# Autodesk Inventor assembly: Central Assembly
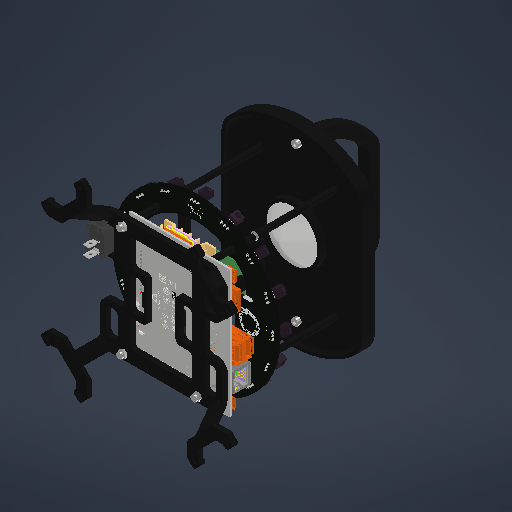
[picture p0: Inventor's stored thumbnail of the model, 512x512]
Saved by Autodesk Inventor 2026.1 (Build 301233020, 233B)
## iProperties
Created: 2026-04-06
Part Number: Central Assembly
Document SubType Name: Assembly
Designer: Bahaa
Mass: 258.249 g
Surface Area: 2094.89 cm^2
Volume: 209.179 cm^3
Density: 1.23458 g/cm^3
Author: Bahaa
## iProperties of the stored document MemberDocs/xZmzij4b1AkjbufniLng3pczf1d
Created: 2026-04-06
Part Number: Central Assembly
Document SubType Name: Assembly
Designer: Bahaa
Mass: 258.233 g
Surface Area: 2094.99 cm^2
Volume: 209.164 cm^3
Density: 1.2346 g/cm^3
Author: Bahaa
## Documents named in this file (20)
- C:\Users\Bahaa\Nextcloud2\CAD\25-26\V2\Central Assembly.iam
- C:\Users\Bahaa\Nextcloud2\CAD\25-26\V2\Center Hub.ipt
- C:\Users\Bahaa\Nextcloud2\CAD\25-26\V2\Parts\675_13541_batuu_dev_kit_top_ass_asm\675_13541_batuu_dev_kit_top_ass_asm.iam
- C:\Users\Bahaa\Nextcloud2\CAD\25-26\V2\Parts\R13-66A-02-BB2.ipt
- C:\Users\Bahaa\Nextcloud2\CAD\25-26\V2\Threaded Rod.ipt
- C:\Users\Bahaa\Documents\Inventor\Content Center Files\R2026\en-US\DIN 985\DIN 985 - M3.ipt
- C:\Users\Bahaa\Documents\Inventor\Content Center Files\R2026\en-US\DIN 934\DIN 934 - M2,5 x 0,45.ipt
- C:\Users\Bahaa\Nextcloud2\CAD\25-26\V2\Rod Housing Jetson.ipt
- C:\Users\Bahaa\Nextcloud2\CAD\25-26\V2\Rod Housing Cam.ipt
- C:\Users\Bahaa\Nextcloud2\CAD\25-26\V2\Camera Bracket.ipt
- C:\Users\Bahaa\Nextcloud2\CAD\25-26\V2\Parts\Kamera.ipt
- C:\Users\Bahaa\Nextcloud2\CAD\25-26\V2\Rod Housing Mirror.ipt
- C:\Users\Bahaa\Nextcloud2\CAD\25-26\V2\Top Cover.ipt
- C:\Users\Bahaa\Nextcloud2\CAD\25-26\V2\Mirror.ipt
- C:\Users\Bahaa\Nextcloud2\CAD\25-26\V2\Handle.ipt
- C:\Users\Bahaa\Documents\Inventor\Content Center Files\R2026\en-US\DIN 912\DIN 912 - M1,6 x 0,35 x 2,5 x 1,625.ipt
- C:\Users\Bahaa\Documents\Inventor\Content Center Files\R2026\en-US\DIN 912\DIN 912 - M3 x 0,5 x 5 x 3,75.ipt
- C:\Users\Bahaa\Nextcloud2\CAD\25-26\V2\Magnet 10x3x2mm.ipt
- C:\Users\Bahaa\Nextcloud2\CAD\25-26\V2\Tag.ipt
- C:\Users\Bahaa\Nextcloud2\CAD\25-26\V2\Boards\IR Board\IR Board\IR Board.iam
## Components (54 placed, 19 different names)
1. Center Hub:1 — Mate:2, Mate:3, Mate:4, Mate:5, Mate:6, Mate:7, Insert:1, Insert:2, Insert:3, Insert:4, Mate:8, Mate:9, Insert:5, Insert:6, Insert:7, Insert:8
2. Camera Bracket:1 — Mate:31, Mate:32, Mate:33, Mate:34, Mate:35, Mate:36, Mate:38, Mate:40, Mate:42, Mate:44
3. Top Cover:1 — Mate:45, Mate:48, Mate:49, Mate:50, Mate:51, Mate:52, Mate:53, Mate:54, Mate:55, Insert:25, Insert:26, Insert:27, Insert:28, Insert:29, Insert:30, Insert:31, Insert:32, Mate:56, Mate:57, Mate:58, Mate:59, Mate:60, Mate:61, Flush:5, Flush:6, Mate:68
4. Handle:1 — Mate:50, Mate:53, Mate:54, Mate:55
5. Mirror:1 — Mate:48, Mate:49
6. Tag:1 — Mate:62, Mate:63, Mate:64, Mate:65, Mate:66, Mate:67, Flush:5, Flush:6, Mate:68
7. IR Board:1 [sub-assembly] — Mate:69, Mate:70, Mate:71
8. Magnet 10x3x2mm:4 — Mate:62, Mate:66, Mate:67
9. Magnet 10x3x2mm:3 — Mate:63, Mate:64, Mate:65
10. Magnet 10x3x2mm:2 — Mate:59, Mate:60, Mate:61
11. Magnet 10x3x2mm:1 — Mate:56, Mate:57, Mate:58
12. DIN 985 - replaced by DIN EN ISO 10511 M3:8 — Insert:32
13. DIN 985 - replaced by DIN EN ISO 10511 M3:7 — Insert:31
14. DIN 985 - replaced by DIN EN ISO 10511 M3:6 — Insert:30
15. DIN 985 - replaced by DIN EN ISO 10511 M3:5 — Insert:29
16. DIN 912 - replaced by DIN EN ISO 4762 M3 x 5:4 — Insert:28
17. DIN 912 - replaced by DIN EN ISO 4762 M3 x 5:3 — Insert:27
18. DIN 912 - replaced by DIN EN ISO 4762 M3 x 5:2 — Insert:26
19. DIN 912 - replaced by DIN EN ISO 4762 M3 x 5:1 — Insert:25
20. DIN 912 - replaced by DIN EN ISO 4762 M1,6 x 2,5:4 — Insert:24
21. DIN 912 - replaced by DIN EN ISO 4762 M1,6 x 2,5:3 — Insert:23
22. DIN 912 - replaced by DIN EN ISO 4762 M1,6 x 2,5:2 — Insert:22
23. DIN 912 - replaced by DIN EN ISO 4762 M1,6 x 2,5:1 — Insert:21
24. DIN 934 - replaced by DIN EN 24032/28673/28674 M2,5:8 — Insert:12
25. DIN 934 - replaced by DIN EN 24032/28673/28674 M2,5:7 — Insert:11, Mate:32
26. DIN 934 - replaced by DIN EN 24032/28673/28674 M2,5:6 — Insert:10
27. DIN 934 - replaced by DIN EN 24032/28673/28674 M2,5:5 — Insert:9
28. DIN 934 - replaced by DIN EN 24032/28673/28674 M2,5:4 — Insert:8
29. DIN 934 - replaced by DIN EN 24032/28673/28674 M2,5:3 — Insert:7, Mate:11
30. DIN 934 - replaced by DIN EN 24032/28673/28674 M2,5:2 — Insert:6
31. DIN 934 - replaced by DIN EN 24032/28673/28674 M2,5:1 — Insert:5
32. DIN 985 - replaced by DIN EN ISO 10511 M3:1 — Insert:1, Flush:2
33. DIN 985 - replaced by DIN EN ISO 10511 M3:2 — Insert:2, Flush:3
34. DIN 985 - replaced by DIN EN ISO 10511 M3:3 — Insert:3, Mate:10, Flush:4
35. DIN 985 - replaced by DIN EN ISO 10511 M3:4 — Insert:4, Flush:1
36. Threaded Rod:1 — Mate:7, Flush:2, Mate:18, Mate:27, Mate:39, Mate:70
37. Threaded Rod:2 — Mate:8, Flush:1, Mate:12, Mate:29, Mate:31, Mate:41, Mate:51
38. Threaded Rod:3 — Mate:9, Flush:3, Mate:19, Mate:22, Mate:28, Mate:37, Mate:52, Mate:71
39. Threaded Rod:4 — Mate:10, Flush:4, Mate:17, Mate:30, Mate:33, Mate:43
40. Rod Housing Mirror:1 — Mate:37, Mate:38
41. Rod Housing Mirror:2 — Mate:39, Mate:40
42. Rod Housing Mirror:3 — Mate:41, Mate:42
43. Rod Housing Mirror:4 — Mate:43, Mate:44, Mate:45
44. Rod Housing Cam:1 — Mate:27, Insert:9
45. Rod Housing Cam:2 — Mate:30, Insert:12
46. Rod Housing Cam:3 — Mate:29, Insert:11
47. Rod Housing Cam:4 — Mate:28, Insert:10
48. Rod Housing Jetson:2 — Mate:14, Mate:17
49. Rod Housing Jetson:3 — Mate:16, Mate:19, Mate:22
50. Rod Housing Jetson:4 — Mate:15, Mate:18
51. Rod Housing Jetson:1 — Mate:12, Mate:13, Mate:69
52. 675_13541_batuu_dev_kit_top_ass_asm:1 [sub-assembly] — Mate:2, Mate:3, Mate:11, Mate:13, Mate:14, Mate:15, Mate:16
53. R13-66A-02-BB2:1 — Mate:4, Mate:5, Mate:6
54. Kamera:1 — Mate:34, Mate:35, Mate:36, Insert:21, Insert:22, Insert:23, Insert:24
## Relationships (92: Mate 62, Insert 24, Flush 6)
- Mate:2: Center Hub:1 ↔ 675_13541_batuu_dev_kit_top_ass_asm:1
- Mate:3: Center Hub:1 ↔ 675_13541_batuu_dev_kit_top_ass_asm:1
- Mate:4 (0.5 mm): Center Hub:1 ↔ R13-66A-02-BB2:1
- Mate:5 (0.2 mm): Center Hub:1 ↔ R13-66A-02-BB2:1
- Mate:6: Center Hub:1 ↔ R13-66A-02-BB2:1
- Mate:7: Center Hub:1 ↔ Threaded Rod:1
- Insert:1: Center Hub:1 ↔ DIN 985 - replaced by DIN EN ISO 10511 M3:1
- Insert:2: Center Hub:1 ↔ DIN 985 - replaced by DIN EN ISO 10511 M3:2
- Insert:3: Center Hub:1 ↔ DIN 985 - replaced by DIN EN ISO 10511 M3:3
- Insert:4: Center Hub:1 ↔ DIN 985 - replaced by DIN EN ISO 10511 M3:4
- Mate:8: Center Hub:1 ↔ Threaded Rod:2
- Flush:1: DIN 985 - replaced by DIN EN ISO 10511 M3:4 ↔ Threaded Rod:2
- Flush:2: DIN 985 - replaced by DIN EN ISO 10511 M3:1 ↔ Threaded Rod:1
- Mate:9: Center Hub:1 ↔ Threaded Rod:3
- Flush:3: DIN 985 - replaced by DIN EN ISO 10511 M3:2 ↔ Threaded Rod:3
- Mate:10: DIN 985 - replaced by DIN EN ISO 10511 M3:3 ↔ Threaded Rod:4
- Flush:4: DIN 985 - replaced by DIN EN ISO 10511 M3:3 ↔ Threaded Rod:4
- Insert:5: Center Hub:1 ↔ DIN 934 - replaced by DIN EN 24032/28673/28674 M2,5:1
- Insert:6: Center Hub:1 ↔ DIN 934 - replaced by DIN EN 24032/28673/28674 M2,5:2
- Insert:7: Center Hub:1 ↔ DIN 934 - replaced by DIN EN 24032/28673/28674 M2,5:3
- Insert:8: Center Hub:1 ↔ DIN 934 - replaced by DIN EN 24032/28673/28674 M2,5:4
- Mate:11: DIN 934 - replaced by DIN EN 24032/28673/28674 M2,5:3 ↔ 675_13541_batuu_dev_kit_top_ass_asm:1
- Mate:12: Threaded Rod:2 ↔ Rod Housing Jetson:1
- Mate:13: Rod Housing Jetson:1 ↔ 675_13541_batuu_dev_kit_top_ass_asm:1
- Mate:14: Rod Housing Jetson:2 ↔ 675_13541_batuu_dev_kit_top_ass_asm:1
- Mate:15: Rod Housing Jetson:4 ↔ 675_13541_batuu_dev_kit_top_ass_asm:1
- Mate:16: Rod Housing Jetson:3 ↔ 675_13541_batuu_dev_kit_top_ass_asm:1
- Mate:17: Threaded Rod:4 ↔ Rod Housing Jetson:2
- Mate:18: Threaded Rod:1 ↔ Rod Housing Jetson:4
- Mate:19: Threaded Rod:3 ↔ Rod Housing Jetson:3
- Mate:22: Threaded Rod:3 ↔ Rod Housing Jetson:3
- Mate:27: Threaded Rod:1 ↔ Rod Housing Cam:1
- Mate:28: Threaded Rod:3 ↔ Rod Housing Cam:4
- Mate:29: Threaded Rod:2 ↔ Rod Housing Cam:3
- Mate:30: Threaded Rod:4 ↔ Rod Housing Cam:2
- Insert:9: DIN 934 - replaced by DIN EN 24032/28673/28674 M2,5:5 ↔ Rod Housing Cam:1
- Insert:10: DIN 934 - replaced by DIN EN 24032/28673/28674 M2,5:6 ↔ Rod Housing Cam:4
- Insert:11: DIN 934 - replaced by DIN EN 24032/28673/28674 M2,5:7 ↔ Rod Housing Cam:3
- Insert:12: DIN 934 - replaced by DIN EN 24032/28673/28674 M2,5:8 ↔ Rod Housing Cam:2
- Mate:31: Camera Bracket:1 ↔ Threaded Rod:2
- Mate:32: Camera Bracket:1 ↔ DIN 934 - replaced by DIN EN 24032/28673/28674 M2,5:7
- Mate:33: Camera Bracket:1 ↔ Threaded Rod:4
- Mate:34: Camera Bracket:1 ↔ Kamera:1
- Mate:35: Camera Bracket:1 ↔ Kamera:1
- Mate:36: Camera Bracket:1 ↔ Kamera:1
- Mate:37: Threaded Rod:3 ↔ Rod Housing Mirror:1
- Mate:38: Camera Bracket:1 ↔ Rod Housing Mirror:1
- Mate:39: Threaded Rod:1 ↔ Rod Housing Mirror:2
- Mate:40: Camera Bracket:1 ↔ Rod Housing Mirror:2
- Mate:41: Threaded Rod:2 ↔ Rod Housing Mirror:3
- Mate:42: Camera Bracket:1 ↔ Rod Housing Mirror:3
- Mate:43: Threaded Rod:4 ↔ Rod Housing Mirror:4
- Mate:44: Camera Bracket:1 ↔ Rod Housing Mirror:4
- Mate:45: Top Cover:1 ↔ Rod Housing Mirror:4
- Mate:48: Top Cover:1 ↔ Mirror:1
- Mate:49: Top Cover:1 ↔ Mirror:1
- Mate:50: Top Cover:1 ↔ Handle:1
- Insert:21: DIN 912 - replaced by DIN EN ISO 4762 M1,6 x 2,5:1 ↔ Kamera:1
- Insert:22: DIN 912 - replaced by DIN EN ISO 4762 M1,6 x 2,5:2 ↔ Kamera:1
- Insert:23: DIN 912 - replaced by DIN EN ISO 4762 M1,6 x 2,5:3 ↔ Kamera:1
- Insert:24: DIN 912 - replaced by DIN EN ISO 4762 M1,6 x 2,5:4 ↔ Kamera:1
- Mate:51: Top Cover:1 ↔ Threaded Rod:2
- Mate:52: Top Cover:1 ↔ Threaded Rod:3
- Mate:53: Top Cover:1 ↔ Handle:1
- Mate:54: Top Cover:1 ↔ Handle:1
- Mate:55: Top Cover:1 ↔ Handle:1
- Insert:25: Top Cover:1 ↔ DIN 912 - replaced by DIN EN ISO 4762 M3 x 5:1
- Insert:26: Top Cover:1 ↔ DIN 912 - replaced by DIN EN ISO 4762 M3 x 5:2
- Insert:27: Top Cover:1 ↔ DIN 912 - replaced by DIN EN ISO 4762 M3 x 5:3
- Insert:28: Top Cover:1 ↔ DIN 912 - replaced by DIN EN ISO 4762 M3 x 5:4
- Insert:29: Top Cover:1 ↔ DIN 985 - replaced by DIN EN ISO 10511 M3:5
- Insert:30: Top Cover:1 ↔ DIN 985 - replaced by DIN EN ISO 10511 M3:6
- Insert:31: Top Cover:1 ↔ DIN 985 - replaced by DIN EN ISO 10511 M3:7
- Insert:32: Top Cover:1 ↔ DIN 985 - replaced by DIN EN ISO 10511 M3:8
- Mate:56: Top Cover:1 ↔ Magnet 10x3x2mm:1
- Mate:57 (0.1 mm): Top Cover:1 ↔ Magnet 10x3x2mm:1
- Mate:58 (0.1 mm): Top Cover:1 ↔ Magnet 10x3x2mm:1
- Mate:59: Top Cover:1 ↔ Magnet 10x3x2mm:2
- Mate:60 (0.1 mm): Top Cover:1 ↔ Magnet 10x3x2mm:2
- Mate:61 (0.1 mm): Top Cover:1 ↔ Magnet 10x3x2mm:2
- Mate:62: Tag:1 ↔ Magnet 10x3x2mm:4
- Mate:63: Tag:1 ↔ Magnet 10x3x2mm:3
- Mate:64 (0.1 mm): Tag:1 ↔ Magnet 10x3x2mm:3
- Mate:65 (0.1 mm): Tag:1 ↔ Magnet 10x3x2mm:3
- Mate:66 (0.1 mm): Tag:1 ↔ Magnet 10x3x2mm:4
- Mate:67 (0.1 mm): Tag:1 ↔ Magnet 10x3x2mm:4
- Flush:5: Top Cover:1 ↔ Tag:1
- Flush:6: Top Cover:1 ↔ Tag:1
- Mate:68: Top Cover:1 ↔ Tag:1
- Mate:69: IR Board:1 ↔ Rod Housing Jetson:1
- Mate:70: IR Board:1 ↔ Threaded Rod:1
- Mate:71: IR Board:1 ↔ Threaded Rod:3
